# Autodesk Inventor assembly: ZŁOŻENIE_OBUDOWA
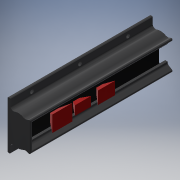
[picture p0: Inventor's stored thumbnail of the model, 180x180]
Saved by Autodesk Inventor 2017 (Build 210142000, 142)
## iProperties
Part Number: ZŁOŻENIE_OBUDOWA
Material: Ogólny
Document SubType Name: Assembly
Designer: patry
Author: patry
## Documents named in this file (4)
- C:\Users\patry\Desktop\realsens\mocowanie\ZŁOŻENIE_OBUDOWA.iam
- C:\Users\patry\Desktop\realsens\SR305_peripheral_assembly_external.iam
- C:\Users\patry\Desktop\realsens\mocowanie\Realsens_basic.ipt
- C:\Users\patry\Desktop\realsens\mocowanie\test_obudowa.ipt
## Components (3 placed, 3 different names)
1. SR305_peripheral_assembly_external:1 [sub-assembly] — Równoległy:1, Równoległy:2, Wstaw:1
2. Realsens_basic:1 — Równoległy:1, Równoległy:2, Wstaw:1, Wstaw:2, Wstaw:3
3. test_obudowa:1 — Wstaw:2, Wstaw:3, Zestawiający:1
## Relationships (6: Insert 3, Flush 2, Mate 1)
- Równoległy:1 [Flush]: SR305_peripheral_assembly_external:1 ↔ Realsens_basic:1
- Równoległy:2 [Flush]: SR305_peripheral_assembly_external:1 ↔ Realsens_basic:1
- Wstaw:1 [Insert]: SR305_peripheral_assembly_external:1 ↔ Realsens_basic:1
- Wstaw:2 [Insert]: Realsens_basic:1 ↔ test_obudowa:1
- Wstaw:3 [Insert]: Realsens_basic:1 ↔ test_obudowa:1
- Zestawiający:1 [Mate]: test_obudowa:1
